# Autodesk Inventor assembly: Assembly1
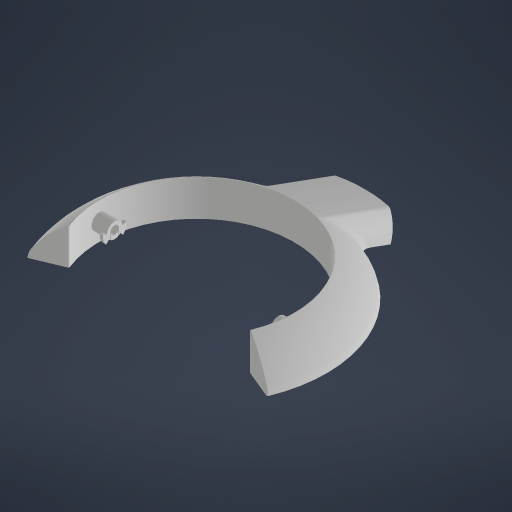
[picture p0: Inventor's stored thumbnail of the model, 512x512]
Saved by Autodesk Inventor 2023 (Build 270158000, 158)
## iProperties
Created: 2021-04-07
Part Number: Assembly1
Document SubType Name: Assembly
Designer: Munsutari
Author: Munsutari
## Documents named in this file (3)
- C:\Users\Munsutari\Desktop\Model Stuff\Siberia 840\Ear Piece Holder.iam
- C:\Users\Munsutari\Desktop\Model Stuff\Siberia 840\Ear Piece Holder.ipt
- C:\Users\Munsutari\Desktop\Model Stuff\Siberia 840\Ear Back Piece.ipt
## Components (2 placed, 2 different names)
1. Ear Piece Holder:1 — Flush:1, Flush:4, Flush:7, Mate:3, Mate:4, Flush:8
2. Ear Back Piece:1 — Flush:1, Flush:4, Flush:7, Mate:3, Mate:4, Flush:8
## Relationships (6: Flush 4, Mate 2)
- Flush:1: Ear Piece Holder:1 ↔ Ear Back Piece:1
- Flush:4: Ear Piece Holder:1 ↔ Ear Back Piece:1
- Flush:7: Ear Piece Holder:1 ↔ Ear Back Piece:1
- Mate:3: Ear Piece Holder:1 ↔ Ear Back Piece:1
- Mate:4: Ear Piece Holder:1 ↔ Ear Back Piece:1
- Flush:8: Ear Piece Holder:1 ↔ Ear Back Piece:1
